# Autodesk Inventor assembly: DinosaurioEnsmablado
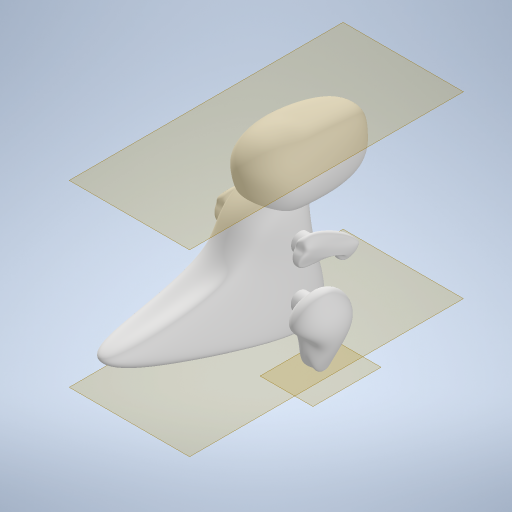
[picture p0: Inventor's stored thumbnail of the model, 512x512]
Saved by Autodesk Inventor 2024.3 (Build 283343000, 343)
## iProperties
Created: 2025-02-09
Part Number: DinosaurioEnsmablado
Document SubType Name: Assembly
Designer: USUARIO
Author: USUARIO
## Documents named in this file (5)
- D:\USUARIO\Documents\Universidad Andres\2024-2\apm\Modelos-Juguetes\Dinosaurio\DinosaurioEnsmablado.iam
- D:\USUARIO\Documents\Universidad Andres\2024-2\apm\Modelos-Juguetes\Dinosaurio\D-Torso.ipt
- D:\USUARIO\Documents\Universidad Andres\2024-2\apm\Modelos-Juguetes\Dinosaurio\D-BrazoDer.ipt
- D:\USUARIO\Documents\Universidad Andres\2024-2\apm\Modelos-Juguetes\Dinosaurio\D-BrazoIzq.ipt
- D:\USUARIO\Documents\Universidad Andres\2024-2\apm\Modelos-Juguetes\Dinosaurio\D-PiernaDer.ipt
## Components (4 placed, 4 different names)
1. D-Torso:1 — Mate:1, Mate:2, Mate:3, Flush:1, Mate:4
2. D-BrazoDer:1 — Mate:1, Mate:2
3. D-BrazoIzq:1 — Mate:3, Flush:1
4. D-PiernaDer:1 — Mate:4
## Relationships (5: Mate 4, Flush 1)
- Mate:1: D-Torso:1 ↔ D-BrazoDer:1
- Mate:2 (7 mm): D-Torso:1 ↔ D-BrazoDer:1
- Mate:3: D-Torso:1 ↔ D-BrazoIzq:1
- Flush:1 (7 mm): D-Torso:1 ↔ D-BrazoIzq:1
- Mate:4: D-Torso:1 ↔ D-PiernaDer:1
